# Autodesk Inventor assembly: ESP32ParasiteMicroscope_v1
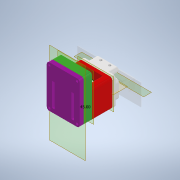
[picture p0: Inventor's stored thumbnail of the model, 180x180]
Saved by Autodesk Inventor 2022 (Build 260153000, 153)
## iProperties
Created: 2022-02-01
Part Number: ESP32ParasiteMicroscope_v1
Document SubType Name: Assembly
Designer: diederichbenedict
Author: diederichbenedict
## Documents named in this file (11)
- C:\Users\Prakash Lab\Documents\Matchboxscope\INVENTOR\ESP32ParasiteMicroscope_v1.iam
- C:\Users\Prakash Lab\Documents\Matchboxscope\INVENTOR\00_chip.ipt
- C:\Users\Prakash Lab\Documents\Matchboxscope\INVENTOR\00_ESP3-CAM.iam
- C:\Users\Prakash Lab\Documents\Matchboxscope\INVENTOR\ESP32ParasiteMicroscope_base_v0.ipt
- C:\Users\Prakash Lab\Documents\Matchboxscope\INVENTOR\ESP32ParasiteMicroscope_top_v0.ipt
- C:\Users\Prakash Lab\Documents\Matchboxscope\INVENTOR\ESP32ParasiteMicroscope_lid_v0.ipt
- C:\Users\diederichbenedict\Documents\Inventor\Content Center Files\R2022\de-DE\DIN 912\DIN 912 - M3 x 0.5 x 25 x 18.ipt
- C:\Users\Prakash Lab\Documents\Matchboxscope\INVENTOR\ESP32ParasiteMicroscope_middle_v1.ipt
- C:\Users\Prakash Lab\Documents\Matchboxscope\INVENTOR\00_CCTV_lens_M12_25mm_5mp.ipt
- C:\Users\Prakash Lab\Documents\Matchboxscope\INVENTOR\ESP32ParasiteMicroscope_m12_knob_v0.ipt
- C:\Users\Prakash Lab\Documents\Matchboxscope\INVENTOR\ESP32ParasiteMicroscope_sample_v1.ipt
## Components (14 placed, 10 different names)
1. ESP32ParasiteMicroscope_base_v0:1 — Fluchtend:3, Fluchtend:4
2. ESP32ParasiteMicroscope_middle_v1:1 — Fluchtend:3, Fluchtend:4, Flush:5
3. ESP32ParasiteMicroscope_top_v0:1 — Angle:1, Flush:5, Flush:7, Flush:8
4. DIN 912 - ersetzt durch DIN EN ISO 4762 M3 x 25:1
5. DIN 912 - ersetzt durch DIN EN ISO 4762 M3 x 25:2
6. DIN 912 - ersetzt durch DIN EN ISO 4762 M3 x 25:3
7. DIN 912 - ersetzt durch DIN EN ISO 4762 M3 x 25:4
8. DIN 912 - ersetzt durch DIN EN ISO 4762 M3 x 25:5
9. 00_ESP3-CAM:1 [sub-assembly] — Insert:7
10. 00_CCTV_lens_M12_25mm_5mp:1 — Insert:7, Mate:1, Flush:6
11. 00_chip:1 — Mate:1, Angle:1, Mate:2
12. ESP32ParasiteMicroscope_lid_v0:1
13. ESP32ParasiteMicroscope_m12_knob_v0:1 — Flush:6
14. ESP32ParasiteMicroscope_sample_v1:1 — Flush:7, Flush:8, Mate:2
## Relationships (10: Flush 6, Mate 2, Insert 1, Angle 1)
- Fluchtend:3 [Flush]: ESP32ParasiteMicroscope_base_v0:1 ↔ ESP32ParasiteMicroscope_middle_v1:1
- Fluchtend:4 [Flush]: ESP32ParasiteMicroscope_base_v0:1 ↔ ESP32ParasiteMicroscope_middle_v1:1
- Insert:7 (12 mm): 00_ESP3-CAM:1 ↔ 00_CCTV_lens_M12_25mm_5mp:1
- Mate:1 (8 mm): 00_CCTV_lens_M12_25mm_5mp:1 ↔ 00_chip:1
- Angle:1 (0 deg): ESP32ParasiteMicroscope_top_v0:1 ↔ 00_chip:1
- Flush:5: ESP32ParasiteMicroscope_middle_v1:1 ↔ ESP32ParasiteMicroscope_top_v0:1
- Flush:6: 00_CCTV_lens_M12_25mm_5mp:1 ↔ ESP32ParasiteMicroscope_m12_knob_v0:1
- Flush:7: ESP32ParasiteMicroscope_top_v0:1 ↔ ESP32ParasiteMicroscope_sample_v1:1
- Flush:8: ESP32ParasiteMicroscope_top_v0:1 ↔ ESP32ParasiteMicroscope_sample_v1:1
- Mate:2: 00_chip:1 ↔ ESP32ParasiteMicroscope_sample_v1:1
